# Autodesk Inventor assembly: linkage_system_test
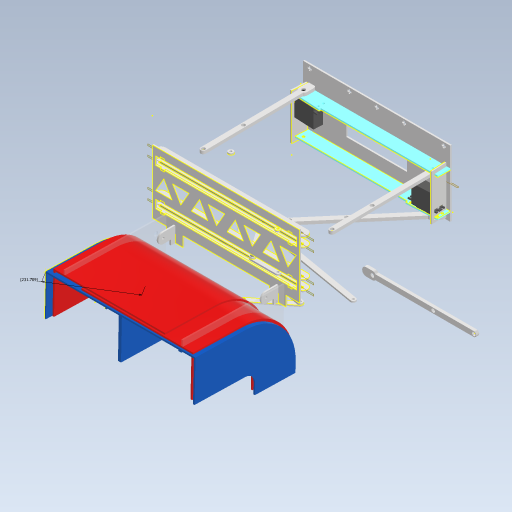
[picture p0: Inventor's stored thumbnail of the model, 512x512]
Saved by Autodesk Inventor 2023 (Build 270158000, 158)
## iProperties
Created: 2023-05-05
Part Number: linkage_system_test
Document SubType Name: Assembly
Designer: 陳詩穎
Author: 陳詩穎
## Documents named in this file (20)
- C:\Users\Johnny Jou\Documents\GitHub\Areo_Rider_Cabin\Expansion\test\linkage_system_test.iam
- C:\Users\Johnny Jou\Documents\GitHub\Areo_Rider_Cabin\Expansion\test\plate_expansion.ipt
- C:\Users\Johnny Jou\Documents\GitHub\Areo_Rider_Cabin\Expansion\test\零件1.ipt
- C:\Users\Johnny Jou\Documents\GitHub\Areo_Rider_Cabin\Expansion\test\零件4.ipt
- C:\Users\Johnny Jou\Documents\GitHub\Areo_Rider_Cabin\Expansion\test\零件5.ipt
- C:\Users\Johnny Jou\Documents\GitHub\Areo_Rider_Cabin\Expansion\test\零件7.ipt
- C:\Users\Johnny Jou\Documents\GitHub\Areo_Rider_Cabin\Airfoil & Nuzzle\nuzzle\nuzzle_v2_0327.ipt
- C:\Users\Johnny Jou\Documents\GitHub\Areo_Rider_Cabin\Airfoil & Nuzzle\nuzzle\nuzzle_v2_0516.ipt
- C:\Users\Johnny Jou\Documents\GitHub\Areo_Rider_Cabin\Airfoil & Nuzzle\nuzzle\nuzzle_v2_0516_2.ipt
- C:\Users\Johnny Jou\Documents\GitHub\Areo_Rider_Cabin\Expansion\test\零件8.ipt
- C:\Users\Johnny Jou\Documents\GitHub\Areo_Rider_Cabin\Expansion\test\零件9.ipt
- C:\Users\Johnny Jou\Documents\GitHub\Areo_Rider_Cabin\Expansion\test\零件10.ipt
- C:\Users\Johnny Jou\Documents\GitHub\Areo_Rider_Cabin\Expansion\test\零件12.ipt
- C:\Users\Johnny Jou\Documents\GitHub\Areo_Rider_Cabin\Expansion\test\adjustable_130.ipt
- C:\Users\Johnny Jou\Documents\GitHub\Areo_Rider_Cabin\Expansion\test\adjustable_80.ipt
- C:\Users\Johnny Jou\Documents\GitHub\Areo_Rider_Cabin\Expansion\test\零件13.ipt
- C:\Users\Johnny Jou\Documents\GitHub\Areo_Rider_Cabin\Expansion\test\bearing_7.ipt
- C:\Users\Johnny Jou\Documents\GitHub\Areo_Rider_Cabin\car\外抓檔\Tower Pro MG996R.ipt
- C:\Users\Johnny Jou\Documents\GitHub\Areo_Rider_Cabin\car\外抓檔\Servo Motor MG996R.ipt
- C:\Users\Johnny Jou\Documents\GitHub\Areo_Rider_Cabin\car\外抓檔\200_forservo.ipt
## Components (37 placed, 19 different names)
1. plate_expansion:1 — 貼合:1, 齊平:1, 貼合:2, 角度:1, 齊平:13, 貼合:255, 齊平:27
2. 零件1:2 — 貼合:1, 齊平:1, 貼合:2, 貼合:49, 貼合:51, 貼合:226, 插入:32, 齊平:28, 貼合:260, 插入:34
3. 零件8:1 — 貼合:49, 貼合:51, 貼合:258
4. 零件12:1 — 插入:7, 貼合:180, 貼合:181, 貼合:182, 貼合:192
5. 零件12:2 — 貼合:177, 貼合:228
6. adjustable_80:2 — 插入:7, 插入:8, 插入:19, 插入:23
7. adjustable_130:1 — 插入:8, 齊平:12
8. adjustable_80:3 — 貼合:178, 插入:15, 貼合:228, 插入:18, 插入:22
9. adjustable_130:2 — 插入:15, 齊平:12
10. 零件4:1 — 貼合:177, 貼合:178, 齊平:8, 齊平:9, 齊平:10, 貼合:187, 貼合:261
11. 零件4:2 — 貼合:183, 齊平:7, 齊平:8, 貼合:189, 貼合:262
12. 零件4:3 — 貼合:180, 貼合:181, 貼合:182, 齊平:9, 貼合:188, 貼合:191
13. 零件4:4 — 齊平:7, 貼合:190, 貼合:193, 貼合:263
14. 零件13:1 — 貼合:183, 貼合:192
15. 零件5:1 — 齊平:10, 貼合:187, 貼合:188, 貼合:189, 貼合:190, 貼合:191, 角度:1, 齊平:13, 齊平:17, 貼合:208, 貼合:209, 貼合:210, 貼合:211, 貼合:212, 貼合:213, 貼合:261, 貼合:262, 貼合:263
16. 零件13:2 — 貼合:193
17. nuzzle_v2_0327:1 — 齊平:17, 貼合:200, 貼合:201
18. nuzzle_v2_0516:1 — 貼合:202, 貼合:203, 貼合:204, 貼合:205, 齊平:18
19. nuzzle_v2_0516_2:1 — 貼合:200, 貼合:201, 貼合:202, 貼合:203, 貼合:206, 齊平:19
20. 零件9:1 — 貼合:204, 貼合:205, 貼合:207, 齊平:18
21. 零件10:1 — 貼合:206, 貼合:207, 齊平:19, 貼合:214
22. 零件7:1 — 貼合:208, 貼合:209, 貼合:210, 貼合:214
23. 零件7:2 — 貼合:211, 貼合:212, 貼合:213
24. 零件8:2 — 貼合:226, 貼合:259, 貼合:260
25. 滾子軸承 GB/T 276-1994 軸承 60000 與 160000 637/4:2 — 插入:18
26. 滾子軸承 GB/T 276-1994 軸承 60000 與 160000 637/4:3 — 插入:19
27. 滾子軸承 GB/T 276-1994 軸承 60000 與 160000 637/4:7 — 插入:23
28. 滾子軸承 GB/T 276-1994 軸承 60000 與 160000 637/4:8 — 插入:22
29. Tower Pro MG996R:1 — 插入:33, 貼合:258, 貼合:264, 貼合:265
30. Tower Pro MG996R:2 — 插入:32, 貼合:259, 貼合:270, 貼合:271
31. 零件1:3 — 貼合:255, 齊平:27, 齊平:28, 插入:33
32. Servo Motor MG996R:1 — 貼合:264, 貼合:265, 貼合:266, 貼合:267, 角度:2
33. 200_forservo:1 — 貼合:266, 貼合:267, 角度:2
34. 200_forservo:2
35. Servo Motor MG996R:2 — 貼合:270, 貼合:271
36. 200_forservo:3
37. 200_forservo:4 — 插入:34
## Relationships (74: Mate 49, Flush 12, Insert 10, Angle 3)
- 貼合:1 [Mate]: plate_expansion:1 ↔ 零件1:2
- 齊平:1 [Flush]: plate_expansion:1 ↔ 零件1:2
- 貼合:2 [Mate]: plate_expansion:1 ↔ 零件1:2
- 貼合:49 [Mate]: 零件1:2 ↔ 零件8:1
- 貼合:51 [Mate]: 零件1:2 ↔ 零件8:1
- 插入:7 [Insert]: 零件12:1 ↔ adjustable_80:2
- 插入:8 [Insert]: adjustable_80:2 ↔ adjustable_130:1
- 貼合:177 [Mate]: 零件12:2 ↔ 零件4:1
- 貼合:178 [Mate]: adjustable_80:3 ↔ 零件4:1
- 貼合:180 [Mate]: 零件12:1 ↔ 零件4:3
- 貼合:181 [Mate]: 零件12:1 ↔ 零件4:3
- 貼合:182 [Mate]: 零件12:1 ↔ 零件4:3
- 貼合:183 [Mate]: 零件4:2 ↔ 零件13:1
- 齊平:7 [Flush]: 零件4:2 ↔ 零件4:4
- 齊平:8 [Flush]: 零件4:1 ↔ 零件4:2
- 齊平:9 [Flush]: 零件4:1 ↔ 零件4:3
- 齊平:10 [Flush]: 零件4:1 ↔ 零件5:1
- 貼合:187 [Mate]: 零件4:1 ↔ 零件5:1
- 貼合:188 [Mate]: 零件4:3 ↔ 零件5:1
- 貼合:189 [Mate]: 零件4:2 ↔ 零件5:1
- 貼合:190 [Mate]: 零件4:4 ↔ 零件5:1
- 貼合:191 [Mate]: 零件4:3 ↔ 零件5:1
- 貼合:192 [Mate]: 零件12:1 ↔ 零件13:1
- 角度:1 [Angle] (0 deg): plate_expansion:1 ↔ 零件5:1
- 插入:15 [Insert]: adjustable_80:3 ↔ adjustable_130:2
- 貼合:193 [Mate]: 零件4:4 ↔ 零件13:2
- 齊平:12 [Flush]: adjustable_130:1 ↔ adjustable_130:2
- 齊平:13 [Flush]: plate_expansion:1 ↔ 零件5:1
- 齊平:17 [Flush] (-2 mm): 零件5:1 ↔ nuzzle_v2_0327:1
- 貼合:200 [Mate]: nuzzle_v2_0327:1 ↔ nuzzle_v2_0516_2:1
- 貼合:201 [Mate]: nuzzle_v2_0327:1 ↔ nuzzle_v2_0516_2:1
- 貼合:202 [Mate]: nuzzle_v2_0516:1 ↔ nuzzle_v2_0516_2:1
- 貼合:203 [Mate]: nuzzle_v2_0516:1 ↔ nuzzle_v2_0516_2:1
- 貼合:204 [Mate]: nuzzle_v2_0516:1 ↔ 零件9:1
- 貼合:205 [Mate]: nuzzle_v2_0516:1 ↔ 零件9:1
- 貼合:206 [Mate]: nuzzle_v2_0516_2:1 ↔ 零件10:1
- 貼合:207 [Mate]: 零件9:1 ↔ 零件10:1
- 齊平:18 [Flush] (-20 mm): nuzzle_v2_0516:1 ↔ 零件9:1
- 齊平:19 [Flush] (20 mm): nuzzle_v2_0516_2:1 ↔ 零件10:1
- 貼合:208 [Mate]: 零件5:1 ↔ 零件7:1
- 貼合:209 [Mate]: 零件5:1 ↔ 零件7:1
- 貼合:210 [Mate]: 零件5:1 ↔ 零件7:1
- 貼合:211 [Mate]: 零件5:1 ↔ 零件7:2
- 貼合:212 [Mate]: 零件5:1 ↔ 零件7:2
- 貼合:213 [Mate]: 零件5:1 ↔ 零件7:2
- 貼合:214 [Mate]: 零件10:1 ↔ 零件7:1
- 貼合:226 [Mate]: 零件1:2 ↔ 零件8:2
- 貼合:228 [Mate]: 零件12:2 ↔ adjustable_80:3
- 插入:18 [Insert]: adjustable_80:3 ↔ 滾子軸承 GB/T 276-1994 軸承 60000 與 160000 637/4:2
- 插入:19 [Insert]: adjustable_80:2 ↔ 滾子軸承 GB/T 276-1994 軸承 60000 與 160000 637/4:3
- 插入:22 [Insert]: adjustable_80:3 ↔ 滾子軸承 GB/T 276-1994 軸承 60000 與 160000 637/4:8
- 插入:23 [Insert]: adjustable_80:2 ↔ 滾子軸承 GB/T 276-1994 軸承 60000 與 160000 637/4:7
- 插入:32 [Insert]: 零件1:2 ↔ Tower Pro MG996R:2
- 貼合:255 [Mate]: plate_expansion:1 ↔ 零件1:3
- 齊平:27 [Flush]: plate_expansion:1 ↔ 零件1:3
- 齊平:28 [Flush]: 零件1:2 ↔ 零件1:3
- 插入:33 [Insert]: Tower Pro MG996R:1 ↔ 零件1:3
- 貼合:258 [Mate]: 零件8:1 ↔ Tower Pro MG996R:1
- 貼合:259 [Mate]: 零件8:2 ↔ Tower Pro MG996R:2
- 貼合:260 [Mate]: 零件1:2 ↔ 零件8:2
- 貼合:261 [Mate]: 零件4:1 ↔ 零件5:1
- 貼合:262 [Mate]: 零件4:2 ↔ 零件5:1
- 貼合:263 [Mate]: 零件4:4 ↔ 零件5:1
- 貼合:264 [Mate]: Tower Pro MG996R:1 ↔ Servo Motor MG996R:1
- 貼合:265 [Mate]: Tower Pro MG996R:1 ↔ Servo Motor MG996R:1
- 貼合:266 [Mate]: Servo Motor MG996R:1 ↔ 200_forservo:1
- 貼合:267 [Mate]: Servo Motor MG996R:1 ↔ 200_forservo:1
- 角度:2 [Angle] (180 deg): Servo Motor MG996R:1 ↔ 200_forservo:1
- [Mate]: Servo Motor MG996R:2 ↔ 200_forservo:3
- [Mate]: Servo Motor MG996R:2 ↔ 200_forservo:3
- [Angle] (180 deg): Servo Motor MG996R:2 ↔ 200_forservo:3
- 貼合:270 [Mate]: Tower Pro MG996R:2 ↔ Servo Motor MG996R:2
- 貼合:271 [Mate]: Tower Pro MG996R:2 ↔ Servo Motor MG996R:2
- 插入:34 [Insert]: 零件1:2 ↔ 200_forservo:4
## Named parameters: d427_d424 = 0 mm, d428_d425 = 0 mm, d429_d426 = 180 deg
